# Autodesk Inventor assembly: SizingCube
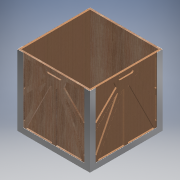
[picture p0: Inventor's stored thumbnail of the model, 180x180]
Saved by Autodesk Inventor 2017.3 (Build 213256000, 256)
## iProperties
Created: 2019-04-26
Part Number: SizingCube
Document SubType Name: Assembly
Designer: guberti
Author: guberti
## Documents named in this file (7)
- C:\Users\guberti\Documents\2019 - 2020 School Year\Inventor\SizingCrate\SizingCube.iam
- C:\Users\guberti\Documents\2019 - 2020 School Year\Inventor\SizingCrate\Bottom.ipt
- C:\Users\guberti\Documents\2019 - 2020 School Year\Inventor\SizingCrate\SizingCrateMinorSide.ipt
- C:\Users\guberti\Documents\2019 - 2020 School Year\Inventor\SizingCrate\SizingCrateMajorSide.ipt
- C:\Users\guberti\Documents\2019 - 2020 School Year\Inventor\SizingCrate\Aluminum Angle Channel-01.ipt
- C:\Users\guberti\Documents\2019 - 2020 School Year\Inventor\SizingCrate\Aluminum Angle Channel.ipt
- C:\Users\guberti\Documents\2019 - 2020 School Year\Inventor\Aluminum Angle Channel-011.ipt
## Components (13 placed, 5 different names)
1. Bottom:1 — Flush:1, Flush:2, Mate:1, Mate:13, Mate:16, Mate:18, Mate:22
2. SizingCrateMinorSide:2 — Flush:1, Flush:2, Mate:1, Flush:5, Flush:6, Mate:3, Flush:7, Mate:4, Flush:9, Flush:13, Flush:14, Mate:9, Mate:15
3. SizingCrateMajorSide:1 — Flush:5, Flush:6, Mate:3, Mate:5, Flush:8, Flush:10, Flush:11, Flush:12, Mate:7, Mate:12
4. Aluminum Angle Channel-01:1 — Flush:15, Mate:8, Mate:9, Mate:17
5. Aluminum Angle Channel-01:2 — Flush:7, Mate:4, Mate:5, Mate:14
6. Aluminum Angle Channel-01:3 — Flush:12, Mate:6, Mate:7, Mate:23
7. Aluminum Angle Channel-01:4 — Flush:16, Mate:10, Mate:11, Mate:20
8. SizingCrateMinorSide:3 — Flush:8, Flush:10, Flush:11, Mate:6, Mate:11, Mate:21
9. SizingCrateMajorSide:2 — Flush:9, Flush:13, Flush:14, Flush:15, Mate:8, Flush:16, Mate:10, Mate:19
10. Aluminum Angle Channel-011:5 — Mate:12, Mate:13, Mate:14
11. Aluminum Angle Channel-011:6 — Mate:15, Mate:16, Mate:17
12. Aluminum Angle Channel-011:7 — Mate:18, Mate:19, Mate:20
13. Aluminum Angle Channel-011:8 — Mate:21, Mate:22, Mate:23
## Relationships (36: Mate 22, Flush 14)
- Flush:1: Bottom:1 ↔ SizingCrateMinorSide:2
- Flush:2: Bottom:1 ↔ SizingCrateMinorSide:2
- Mate:1: Bottom:1 ↔ SizingCrateMinorSide:2
- Flush:5: SizingCrateMinorSide:2 ↔ SizingCrateMajorSide:1
- Flush:6: SizingCrateMinorSide:2 ↔ SizingCrateMajorSide:1
- Mate:3: SizingCrateMinorSide:2 ↔ SizingCrateMajorSide:1
- Flush:7: SizingCrateMinorSide:2 ↔ Aluminum Angle Channel-01:2
- Mate:4: SizingCrateMinorSide:2 ↔ Aluminum Angle Channel-01:2
- Mate:5: SizingCrateMajorSide:1 ↔ Aluminum Angle Channel-01:2
- Flush:8: SizingCrateMajorSide:1 ↔ SizingCrateMinorSide:3
- Flush:9: SizingCrateMinorSide:2 ↔ SizingCrateMajorSide:2
- Flush:10: SizingCrateMajorSide:1 ↔ SizingCrateMinorSide:3
- Flush:11: SizingCrateMajorSide:1 ↔ SizingCrateMinorSide:3
- Flush:12: SizingCrateMajorSide:1 ↔ Aluminum Angle Channel-01:3
- Mate:6: Aluminum Angle Channel-01:3 ↔ SizingCrateMinorSide:3
- Mate:7: SizingCrateMajorSide:1 ↔ Aluminum Angle Channel-01:3
- Flush:13: SizingCrateMinorSide:2 ↔ SizingCrateMajorSide:2
- Flush:14: SizingCrateMinorSide:2 ↔ SizingCrateMajorSide:2
- Flush:15: Aluminum Angle Channel-01:1 ↔ SizingCrateMajorSide:2
- Mate:8: Aluminum Angle Channel-01:1 ↔ SizingCrateMajorSide:2
- Mate:9: SizingCrateMinorSide:2 ↔ Aluminum Angle Channel-01:1
- Flush:16: Aluminum Angle Channel-01:4 ↔ SizingCrateMajorSide:2
- Mate:10: Aluminum Angle Channel-01:4 ↔ SizingCrateMajorSide:2
- Mate:11: Aluminum Angle Channel-01:4 ↔ SizingCrateMinorSide:3
- Mate:12: SizingCrateMajorSide:1 ↔ Aluminum Angle Channel-011:5
- Mate:13: Bottom:1 ↔ Aluminum Angle Channel-011:5
- Mate:14: Aluminum Angle Channel-01:2 ↔ Aluminum Angle Channel-011:5
- Mate:15: SizingCrateMinorSide:2 ↔ Aluminum Angle Channel-011:6
- Mate:16: Bottom:1 ↔ Aluminum Angle Channel-011:6
- Mate:17: Aluminum Angle Channel-01:1 ↔ Aluminum Angle Channel-011:6
- Mate:18: Bottom:1 ↔ Aluminum Angle Channel-011:7
- Mate:19: SizingCrateMajorSide:2 ↔ Aluminum Angle Channel-011:7
- Mate:20: Aluminum Angle Channel-01:4 ↔ Aluminum Angle Channel-011:7
- Mate:21: SizingCrateMinorSide:3 ↔ Aluminum Angle Channel-011:8
- Mate:22: Bottom:1 ↔ Aluminum Angle Channel-011:8
- Mate:23: Aluminum Angle Channel-01:3 ↔ Aluminum Angle Channel-011:8
